# Autodesk Inventor assembly: assembl nozzle
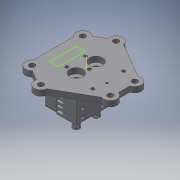
[picture p0: Inventor's stored thumbnail of the model, 180x180]
Saved by Autodesk Inventor 2016 SP1 (Build 200210100, 210)
## iProperties
Created: 2016-04-15
Part Number: assembl nozzle
Document SubType Name: Assembly
Designer: ubik
Author: ubik
## Documents named in this file (5)
- E:\GitHub\kossel-XXL\assembl nozzle.iam
- E:\GitHub\kossel-XXL\efector.ipt
- E:\GitHub\kossel-XXL\nozzel heat sink.ipt
- E:\GitHub\kossel-XXL\nozzle throat.ipt
- E:\GitHub\kossel-XXL\30x30 fan cooler.ipt
## Components (5 placed, 4 different names)
1. efector:1 — Mate:5, Mate:6, Mate:7
2. nozzel heat sink:1 — Mate:1, Mate:2, Mate:3, Mate:4, Mate:5, Mate:6, Mate:7, Mate:8, Flush:1, Flush:2
3. nozzle throat:1 — Mate:1, Mate:3
4. nozzle throat:2 — Mate:2, Mate:4
5. 30x30 fan cooler:1 — Mate:8, Flush:1, Flush:2
## Relationships (10: Mate 8, Flush 2)
- Mate:1: nozzel heat sink:1 ↔ nozzle throat:1
- Mate:2: nozzel heat sink:1 ↔ nozzle throat:2
- Mate:3: nozzel heat sink:1 ↔ nozzle throat:1
- Mate:4: nozzel heat sink:1 ↔ nozzle throat:2
- Mate:5: efector:1 ↔ nozzel heat sink:1
- Mate:6: efector:1 ↔ nozzel heat sink:1
- Mate:7: efector:1 ↔ nozzel heat sink:1
- Mate:8: nozzel heat sink:1 ↔ 30x30 fan cooler:1
- Flush:1: nozzel heat sink:1 ↔ 30x30 fan cooler:1
- Flush:2: nozzel heat sink:1 ↔ 30x30 fan cooler:1
